# Autodesk Inventor assembly: ASY NDM_VOS pillar 1
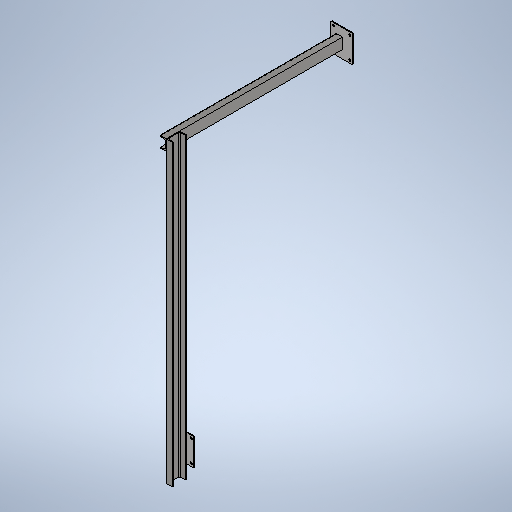
[picture p0: Inventor's stored thumbnail of the model, 512x512]
Saved by Autodesk Inventor 2025 (Build 290162010, 162A)
## iProperties
Created: 2025-11-03
Part Number: ASY NDM_VOS pillar 1
Document SubType Name: Assembly
Designer: admin
Author: admin
## Documents named in this file (4)
- C:\Users\admin\Yandex.Disk\home pc\Inventor\NDM-VOS_powder_hopper\400 tube\ASY NDM_VOS pillar 1.iam
- C:\Users\admin\Yandex.Disk\home pc\Inventor\NDM-VOS_powder_hopper\400 tube\NDM-VOS pillar 1 ch 1.ipt
- C:\Users\admin\Yandex.Disk\home pc\Inventor\NDM-VOS_powder_hopper\400 tube\Part2.ipt
- C:\Users\admin\Yandex.Disk\home pc\Inventor\NDM-VOS_powder_hopper\400 tube\NDM-VOS pillar 1 ch 2.ipt
## Components (4 placed, 3 different names)
1. NDM-VOS pillar 1 ch 1:1 — Rigid:1, Rigid:2
2. Part2:1 — Rigid:1
3. NDM-VOS pillar 1 ch 2:1 — Rigid:2, Rigid:3
4. Part2:2 — Rigid:3
## Relationships (3: WeldJoint 3)
- Rigid:1 [WeldJoint] (100 mm): NDM-VOS pillar 1 ch 1:1 ↔ Part2:1
- Rigid:2 [WeldJoint]: NDM-VOS pillar 1 ch 1:1 ↔ NDM-VOS pillar 1 ch 2:1
- Rigid:3 [WeldJoint]: NDM-VOS pillar 1 ch 2:1 ↔ Part2:2
